# Autodesk Inventor assembly: CamProfile_Trans_offset_roller_Cycloid
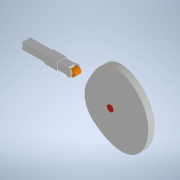
[picture p0: Inventor's stored thumbnail of the model, 180x180]
Saved by Autodesk Inventor 2022 (Build 260153000, 153)
## iProperties
Created: 2023-03-23
Part Number: CamProfile_Trans_offset_roller_Cycloid
Document SubType Name: Assembly
Designer: JOU
Author: JOU
## Documents named in this file (6)
- C:\Users\JOU\Desktop\git\Special-project\CamProfile_Trans_offset_roller_Cycloid.iam
- C:\Users\JOU\Desktop\git\Special-project\axis.ipt
- C:\Users\JOU\Desktop\git\Special-project\CamProfile_Trans_offset_roller_Cycloid.ipt
- C:\Users\JOU\Desktop\git\Special-project\axis_rf_fix.ipt
- C:\Users\JOU\Desktop\git\Special-project\axis_rf.ipt
- C:\Users\JOU\Desktop\git\Special-project\rf.ipt
## Components (5 placed, 5 different names)
1. axis:1 — 插入:1
2. CamProfile_Trans_offset_roller_Cycloid:1 — 插入:1
3. axis_rf_fix:1 — 貼合:1, 貼合:2, 貼合:3, 貼合:4, 齊平:1
4. axis_rf:1 — 插入:2, 貼合:1, 貼合:2
5. rf:1 — 插入:2
## Relationships (7: Mate 4, Insert 2, Flush 1)
- 插入:1 [Insert]: axis:1 ↔ CamProfile_Trans_offset_roller_Cycloid:1
- 插入:2 [Insert]: axis_rf:1 ↔ rf:1
- 貼合:1 [Mate]: axis_rf_fix:1 ↔ axis_rf:1
- 貼合:2 [Mate]: axis_rf_fix:1 ↔ axis_rf:1
- 貼合:3 [Mate] (6.25 mm): axis_rf_fix:1
- 貼合:4 [Mate] (12 mm): axis_rf_fix:1
- 齊平:1 [Flush] (80 mm): axis_rf_fix:1
